# Autodesk Inventor assembly: Gooseneck Model-1
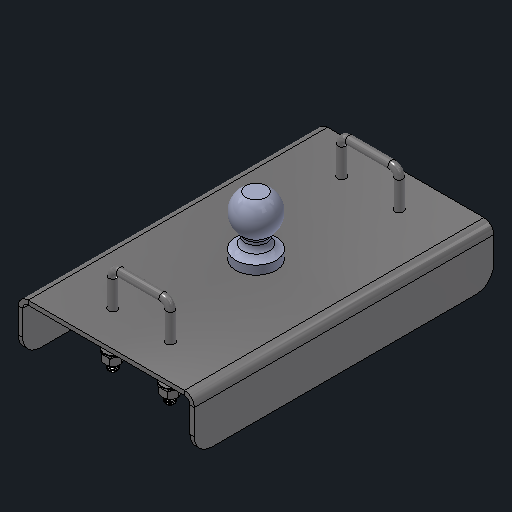
[picture p0: Inventor's stored thumbnail of the model, 512x512]
Saved by Autodesk Inventor 2025.1 (Build 291241000, 241)
## iProperties
Created: 2026-02-16
Part Number: Gooseneck Model-1
Document SubType Name: Assembly
Designer: Desktop -24
encoded128: ÌStandard (in)rÎ
Family: ASSEMBLY
Author: Desktop -24
## Documents named in this file (5)
- F:\OneDrive - nLeague Technologies Private Limited\Desktop\Sharath Chandra\Goose Neck\Gooseneck Model-1\Gooseneck Model-1.iam
- F:\OneDrive - nLeague Technologies Private Limited\Desktop\Sharath Chandra\Goose Neck\Gooseneck Model-1\Gooseneck Model-1 Sheet-1.ipt
- F:\OneDrive - nLeague Technologies Private Limited\Desktop\Sharath Chandra\Goose Neck\Gooseneck Model-1\Gooseneck Model-1 Ball.ipt
- F:\OneDrive - nLeague Technologies Private Limited\Desktop\Sharath Chandra\Goose Neck\Gooseneck Model-1\Gooseneck Model-1 Sheet-2.ipt
- F:\OneDrive - nLeague Technologies Private Limited\Desktop\Sharath Chandra\Goose Neck\Gooseneck Model-1\Gooseneck Model-1 Hitch Clamp.ipt
## Components (5 placed, 4 different names)
1. Gooseneck Model-1 Sheet-1:1 — Mate:1, Mate:2, Mate:3, Mate:5, Mate:6, Mate:7, Mate:8, Mate:9
2. Gooseneck Model-1 Ball:1 — Mate:1, Mate:2, Mate:4
3. Gooseneck Model-1 Sheet-2:1 — Mate:3, Mate:4
4. Gooseneck Model-1 Hitch Clamp:1 — Mate:5, Mate:6, Flush:1
5. Gooseneck Model-1 Hitch Clamp:2 — Mate:7, Mate:8, Flush:1, Mate:9
## Relationships (10: Mate 9, Flush 1)
- Mate:1: Gooseneck Model-1 Sheet-1:1 ↔ Gooseneck Model-1 Ball:1
- Mate:2 (12.7 mm): Gooseneck Model-1 Sheet-1:1 ↔ Gooseneck Model-1 Ball:1
- Mate:3: Gooseneck Model-1 Sheet-1:1 ↔ Gooseneck Model-1 Sheet-2:1
- Mate:4: Gooseneck Model-1 Ball:1 ↔ Gooseneck Model-1 Sheet-2:1
- Mate:5: Gooseneck Model-1 Sheet-1:1 ↔ Gooseneck Model-1 Hitch Clamp:1
- Mate:6: Gooseneck Model-1 Sheet-1:1 ↔ Gooseneck Model-1 Hitch Clamp:1
- Mate:7: Gooseneck Model-1 Sheet-1:1 ↔ Gooseneck Model-1 Hitch Clamp:2
- Mate:8: Gooseneck Model-1 Sheet-1:1 ↔ Gooseneck Model-1 Hitch Clamp:2
- Flush:1: Gooseneck Model-1 Hitch Clamp:1 ↔ Gooseneck Model-1 Hitch Clamp:2
- Mate:9 (50.8 mm): Gooseneck Model-1 Sheet-1:1 ↔ Gooseneck Model-1 Hitch Clamp:2
